# Autodesk Inventor assembly: Assieme completo - Trasporto Taglio
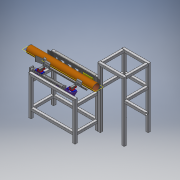
[picture p0: Inventor's stored thumbnail of the model, 180x180]
Saved by Autodesk Inventor 2018 (Build 220112000, 112)
## iProperties
Created: 2020-06-01
Part Number: Assieme completo - Trasporto Taglio
Material: Generico
Document SubType Name: Assembly
Designer: Francesco
Author: Francesco
## Documents named in this file (3)
- C:\Users\Francesco\no-brim\Meccanica\Progetto Inventor no-brim\Assiemi\Assieme completo - Trasporto Taglio.iam
- C:\Users\Francesco\no-brim\Meccanica\Progetto Inventor no-brim\Assiemi\Assieme 1 - Trasporto.iam
- C:\Users\Francesco\no-brim\Meccanica\Progetto Inventor no-brim\Assiemi\Assieme 2 - Taglio.iam
## Components (2 placed, 2 different names)
1. Assieme 1 - Trasporto:1 [sub-assembly] — Allineato:1, Allineato:2, Coincidente:1
2. Assieme 2 - Taglio:1 [sub-assembly] — Allineato:1, Allineato:2, Coincidente:1
## Relationships (3: Flush 2, Mate 1)
- Allineato:1 [Flush]: Assieme 1 - Trasporto:1 ↔ Assieme 2 - Taglio:1
- Allineato:2 [Flush]: Assieme 1 - Trasporto:1 ↔ Assieme 2 - Taglio:1
- Coincidente:1 [Mate]: Assieme 1 - Trasporto:1 ↔ Assieme 2 - Taglio:1
